# Autodesk Inventor assembly: mainasm
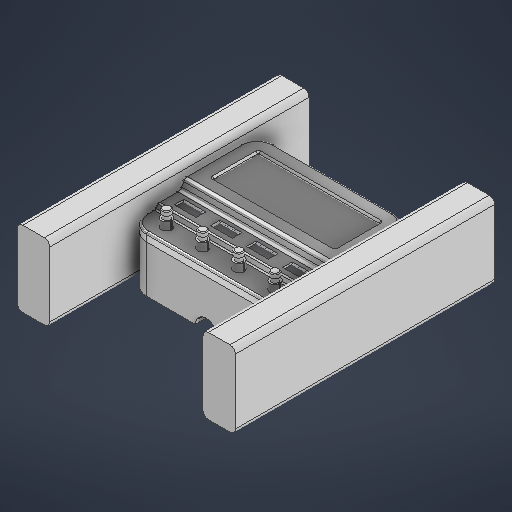
[picture p0: Inventor's stored thumbnail of the model, 512x512]
Saved by Autodesk Inventor 2025.3 (Build 293356000, 356)
## iProperties
Created: 2026-02-28
Part Number: mainasm
Document SubType Name: Assembly
Designer: Lemon
Author: Lemon
## Documents named in this file (7)
- C:\Users\Lemon\Documents\Inventor\SmartBreaker\mainasm.iam
- C:\Users\Lemon\Documents\Inventor\SmartBreaker\BreakerFront.ipt
- C:\Users\Lemon\Documents\Inventor\SmartBreaker\COTS\ar70736.ipt
- C:\Users\Lemon\Documents\Inventor\SmartBreaker\COTS\OLED_0.91_128x32\OLED_0.91_128x32.iam
- C:\Users\Lemon\Documents\Inventor\SmartBreaker\COTS\CrowPanel ESP32 5.79” E-paper HMI Display\CrowPanel ESP32 5.79” E-paper HMI Display\CrowPanel ESP32 5.79” E-paper HMI Display.iam
- C:\Users\Lemon\Documents\Inventor\SmartBreaker\BreakerRear.ipt
- C:\Users\Lemon\Documents\Inventor\SmartBreaker\2by4mog.ipt
## Components (13 placed, 6 different names)
1. BreakerFront:1 — Mate:1, Mate:2, Angle:1, Mate:3, Angle:2, Angle:3, Angle:4, Mate:4, Mate:5, Mate:6, Mate:7, Mate:8, Mate:9, Mate:10, Mate:11, Mate:12, Mate:13, Mate:14, Mate:15, Mate:16
2. ar70736:1 — Mate:2, Angle:1, Mate:3
3. OLED_0.91_128x32:1 [sub-assembly] — Mate:10
4. CrowPanel ESP32 5.79” E-paper HMI Display:1 [sub-assembly] — Mate:1
5. OLED_0.91_128x32:2 [sub-assembly] — Mate:11
6. OLED_0.91_128x32:3 [sub-assembly] — Mate:12
7. OLED_0.91_128x32:4 [sub-assembly] — Mate:13
8. ar70736:2 — Angle:2, Mate:6, Mate:7
9. ar70736:3 — Angle:3, Mate:5, Mate:8
10. ar70736:4 — Angle:4, Mate:4, Mate:9
11. BreakerRear:1 — Mate:14, Mate:15, Mate:16, Mate:17, Mate:18, Mate:19, Mate:20
12. 2by4mog:1 — Mate:17, Mate:18, Flush:1
13. 2by4mog:2 — Mate:19, Mate:20, Flush:1
## Relationships (25: Mate 20, Angle 4, Flush 1)
- Mate:1: BreakerFront:1 ↔ CrowPanel ESP32 5.79” E-paper HMI Display:1
- Mate:2: BreakerFront:1 ↔ ar70736:1
- Angle:1 (180 deg): BreakerFront:1 ↔ ar70736:1
- Mate:3: BreakerFront:1 ↔ ar70736:1
- Angle:2 (180 deg): BreakerFront:1 ↔ ar70736:2
- Angle:3 (180 deg): BreakerFront:1 ↔ ar70736:3
- Angle:4 (180 deg): BreakerFront:1 ↔ ar70736:4
- Mate:4: BreakerFront:1 ↔ ar70736:4
- Mate:5: BreakerFront:1 ↔ ar70736:3
- Mate:6: BreakerFront:1 ↔ ar70736:2
- Mate:7: BreakerFront:1 ↔ ar70736:2
- Mate:8: BreakerFront:1 ↔ ar70736:3
- Mate:9: BreakerFront:1 ↔ ar70736:4
- Mate:10: BreakerFront:1 ↔ OLED_0.91_128x32:1
- Mate:11: BreakerFront:1 ↔ OLED_0.91_128x32:2
- Mate:12: BreakerFront:1 ↔ OLED_0.91_128x32:3
- Mate:13: BreakerFront:1 ↔ OLED_0.91_128x32:4
- Mate:14: BreakerFront:1 ↔ BreakerRear:1
- Mate:15: BreakerFront:1 ↔ BreakerRear:1
- Mate:16: BreakerFront:1 ↔ BreakerRear:1
- Mate:17: BreakerRear:1 ↔ 2by4mog:1
- Mate:18: BreakerRear:1 ↔ 2by4mog:1
- Mate:19: BreakerRear:1 ↔ 2by4mog:2
- Mate:20: BreakerRear:1 ↔ 2by4mog:2
- Flush:1: 2by4mog:1 ↔ 2by4mog:2
